# Autodesk Inventor assembly: Assy_test
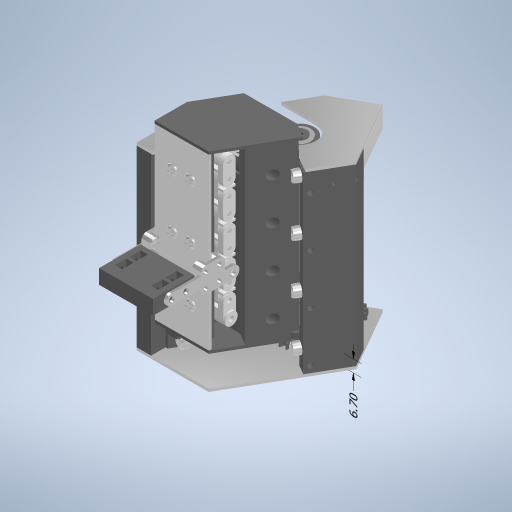
[picture p0: Inventor's stored thumbnail of the model, 512x512]
Saved by Autodesk Inventor 2024.1 (Build 281209000, 209)
## iProperties
Created: 2025-01-17
Part Number: Assy_test
Document SubType Name: Assembly
Designer: hibik
Author: hibik
## Documents named in this file (6)
- C:\Users\hibik\Documents\Robomech\RESCUE\ORCA\hard\fork\right\Assy_test.iam
- C:\Users\hibik\Documents\Robomech\RESCUE\ORCA\hard\fork\right\screw.iam
- C:\Users\hibik\Documents\Robomech\RESCUE\ORCA\hard\std_parts\motor_6V_60RPM.ipt
- C:\Users\hibik\Documents\Robomech\RESCUE\ORCA\hard\fork\right\screw_gear_under.ipt
- C:\Users\hibik\Documents\Robomech\RESCUE\ORCA\hard\fork\right\base.iam
- C:\Users\hibik\Documents\Robomech\RESCUE\ORCA\hard\fork\right\rail.iam
## Components (5 placed, 5 different names)
1. screw:1 [sub-assembly] — 挿入:1
2. motor_6V_60RPM:1 — 挿入:3
3. screw_gear_under:1 — 挿入:2, 挿入:3
4. base:1 [sub-assembly] — 挿入:1, 挿入:2, 正接:1, 正接:2
5. rail:1 [sub-assembly] — 正接:1, 正接:2
## Relationships (5: Insert 3, Tangent 2)
- 挿入:1 [Insert]: screw:1 ↔ base:1
- 挿入:2 [Insert]: screw_gear_under:1 ↔ base:1
- 挿入:3 [Insert]: motor_6V_60RPM:1 ↔ screw_gear_under:1
- 正接:1 [Tangent]: base:1 ↔ rail:1
- 正接:2 [Tangent]: base:1 ↔ rail:1
